# Autodesk Inventor assembly: ASSEMBLY_Visual_inspection_tray_with_rear_mount
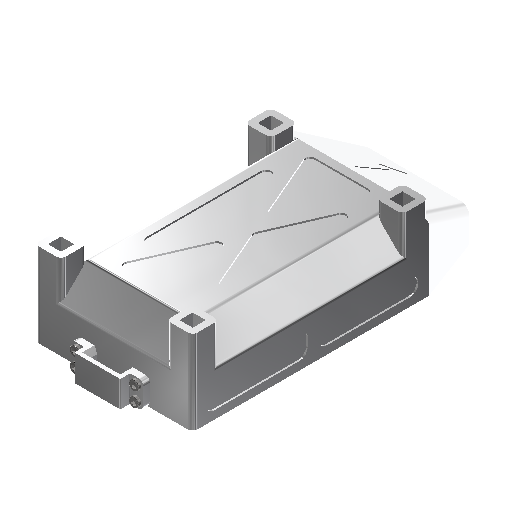
[picture p0: Inventor's stored thumbnail of the model, 512x512]
Saved by Autodesk Inventor 2025 (Build 290162010, 162A)
## iProperties
Created: 2018-09-18
Part Number: ASSEMBLY_Visual_inspection_tray_with_rear_mount
Document SubType Name: Assembly
Designer: Andrzej
Mass: 43.0897 g
Surface Area: 178.201 cm^2
Volume: 15.862 cm^3
Density: 2.71653 g/cm^3
Author: Andrzej
## Documents named in this file (4)
- D:\_ANDRZEJ_LACZEWSKI\_OTHER\MECH - My entry for the NASA Lunar Sampling System Design Challenge\MCAD\1_REV1\ASSEMBLY_MAIN_REVA\ASSEMBLY_Visual_inspection_tray_with_rear_mount.iam
- D:\_ANDRZEJ_LACZEWSKI\_OTHER\MECH - My entry for the NASA Lunar Sampling System Design Challenge\MCAD\1_REV1\ASSEMBLY_MAIN_REVA\Visual inspection tray v2.ipt
- D:\_ANDRZEJ_LACZEWSKI\_OTHER\MECH - My entry for the NASA Lunar Sampling System Design Challenge\MCAD\1_REV1\ASSEMBLY_MAIN_REVA\Visual inspection tray bucket mount.ipt
- D:\_ANDRZEJ_LACZEWSKI\_OTHER\MECH - My entry for the NASA Lunar Sampling System Design Challenge\MCAD\1_REV1\ASSEMBLY_MAIN_REVA\M1,6x3,5.ipt
## Components (6 placed, 3 different names)
1. Visual inspection tray v2:1 — Mate:13, Flush:1, Flush:2
2. Visual inspection tray bucket mount:1 — Mate:13, Flush:1, Flush:2, Mate:14, Mate:15, Mate:16, Mate:17, Mate:18, Mate:19, Mate:20, Mate:21
3. M1,6x3,5:1 — Mate:14, Mate:18
4. M1,6x3,5:2 — Mate:15, Mate:19
5. M1,6x3,5:3 — Mate:16, Mate:20
6. M1,6x3,5:4 — Mate:17, Mate:21
## Relationships (11: Mate 9, Flush 2)
- Mate:13: Visual inspection tray v2:1 ↔ Visual inspection tray bucket mount:1
- Flush:1: Visual inspection tray v2:1 ↔ Visual inspection tray bucket mount:1
- Flush:2 (13 mm): Visual inspection tray v2:1 ↔ Visual inspection tray bucket mount:1
- Mate:14: Visual inspection tray bucket mount:1 ↔ M1,6x3,5:1
- Mate:15: Visual inspection tray bucket mount:1 ↔ M1,6x3,5:2
- Mate:16: Visual inspection tray bucket mount:1 ↔ M1,6x3,5:3
- Mate:17: Visual inspection tray bucket mount:1 ↔ M1,6x3,5:4
- Mate:18: Visual inspection tray bucket mount:1 ↔ M1,6x3,5:1
- Mate:19: Visual inspection tray bucket mount:1 ↔ M1,6x3,5:2
- Mate:20: Visual inspection tray bucket mount:1 ↔ M1,6x3,5:3
- Mate:21: Visual inspection tray bucket mount:1 ↔ M1,6x3,5:4
